# Autodesk Inventor assembly: Arm
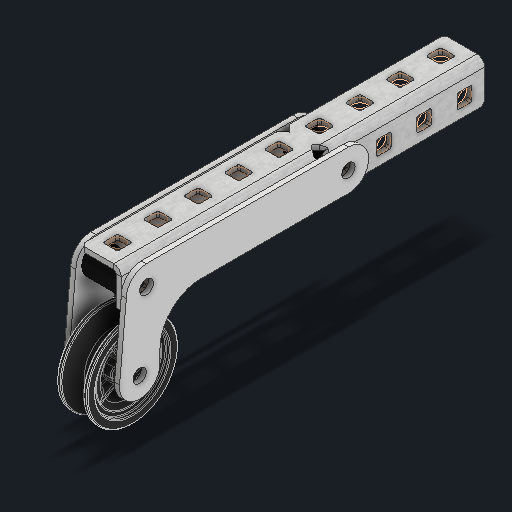
[picture p0: Inventor's stored thumbnail of the model, 512x512]
Saved by Autodesk Inventor 2025.1 (Build 291241000, 241)
## iProperties
Created: 2024-10-24
Part Number: Arm
Document SubType Name: Assembly
Designer: avere
Author: avere
## Documents named in this file (7)
- C:\Users\avere\VEX\High Stakes\CAD\V2\Hang\Arm.iam
- C:\Users\avere\VEX\High Stakes\CAD\ROBOPROS-CAD-Inventor\Structure\Angle\Aluminum 1x1\Alu Angle 1x1x9.ipt
- C:\Users\avere\VEX\High Stakes\CAD\ROBOPROS-CAD-Inventor\Motion\Spacers\Spacer Nylon .375 OD\NSpacer .375 OD x .500.ipt
- C:\Users\avere\VEX\High Stakes\CAD\ROBOPROS-CAD-Inventor\Motion\Spacers\Spacer Nylon .375 OD.ipt
- C:\Users\avere\VEX\High Stakes\CAD\V2\Hang\Custom Parts\Passive Gusset.ipt
- C:\Users\avere\VEX\High Stakes\CAD\ROBOPROS-CAD-Inventor\Motion\Pulley.ipt
- C:\Users\avere\VEX\High Stakes\CAD\ROBOPROS-CAD-Inventor\Structure\Hardware\Nut Keps.ipt
## Components (7 placed, 5 different names)
1. Alu Angle 1x1x9:1 — Insert:1, Insert:2, Insert:3, Mate:1
2. NSpacer .375 OD x .500:1 — Insert:2, Mate:2
3. NSpacer .375 OD x .500:2 — Insert:1, Insert:4
4. Passive Gusset:1 — Insert:3, Mate:1
5. Passive Gusset:2 — Insert:4, Mate:2, Insert:5
6. Pulley:1 — Insert:6
7. Nut Keps:1 — Insert:5, Insert:6
## Relationships (8: Insert 6, Mate 2)
- Insert:1: Alu Angle 1x1x9:1 ↔ NSpacer .375 OD x .500:2
- Insert:2: Alu Angle 1x1x9:1 ↔ NSpacer .375 OD x .500:1
- Insert:3: Alu Angle 1x1x9:1 ↔ Passive Gusset:1
- Mate:1: Alu Angle 1x1x9:1 ↔ Passive Gusset:1
- Insert:4: NSpacer .375 OD x .500:2 ↔ Passive Gusset:2
- Mate:2: NSpacer .375 OD x .500:1 ↔ Passive Gusset:2
- Insert:5: Passive Gusset:2 ↔ Nut Keps:1
- Insert:6 (0.3969 mm): Pulley:1 ↔ Nut Keps:1
